# Autodesk Inventor assembly: platform
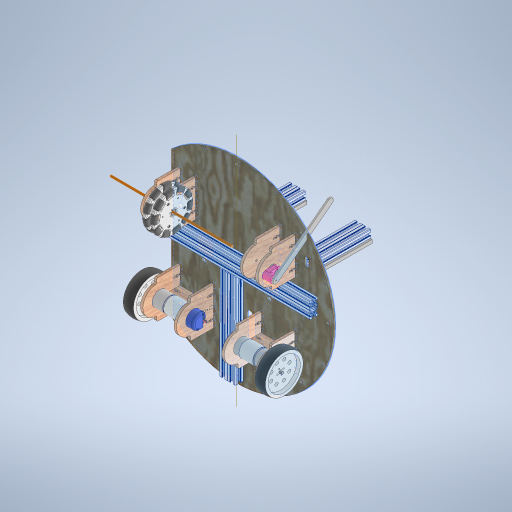
[picture p0: Inventor's stored thumbnail of the model, 512x512]
Saved by Autodesk Inventor 2023.1 (Build 271208000, 208)
## iProperties
Created: 2023-03-13
Part Number: platform
Document SubType Name: Assembly
Designer: User
Author: User
## Documents named in this file (24)
- C:\Users\DELL\reposGitHub\Cheburashka\Cheburashka_construction\platform\platform.iam
- C:\Users\DELL\reposGitHub\Cheburashka\Cheburashka_construction\platform\Osn. platform.ipt
- C:\Users\DELL\reposGitHub\Cheburashka\Cheburashka_construction\platform\motor1.ipt
- C:\Users\DELL\reposGitHub\Cheburashka\Cheburashka_construction\platform\motor2.ipt
- C:\Users\DELL\reposGitHub\Cheburashka\Cheburashka_construction\platform\motor3.ipt
- C:\Users\DELL\reposGitHub\Cheburashka\Cheburashka_construction\platform\wheel1.ipt
- C:\Users\DELL\reposGitHub\Cheburashka\Cheburashka_construction\platform\44260_txm torquenado dc motor_MIR2.ipt
- C:\Users\DELL\reposGitHub\Cheburashka\Cheburashka_construction\platform\36466_txm-4 inch omni wheel.ipt
- C:\Users\DELL\reposGitHub\Cheburashka\Cheburashka_construction\platform\39055_txm-4 inch wheel_MIR1.ipt
- C:\Users\DELL\reposGitHub\Cheburashka\Cheburashka_construction\platform\motor1_MIR3.ipt
- C:\Users\DELL\reposGitHub\Cheburashka\Cheburashka_construction\platform\motor2_MIR3.ipt
- C:\Users\DELL\reposGitHub\Cheburashka\Cheburashka_construction\platform\motor3_MIR3.ipt
- C:\Users\DELL\reposGitHub\Cheburashka\Cheburashka_construction\platform\44260_txm torquenado dc motor_MIR2_MIR.ipt
- C:\Users\DELL\reposGitHub\Cheburashka\Cheburashka_construction\platform\wheel1_MIR.ipt
- C:\Users\DELL\reposGitHub\Cheburashka\Cheburashka_construction\platform\36466_txm-4 inch omni wheel_MIR2.ipt
- C:\Users\DELL\reposGitHub\Cheburashka\Cheburashka_construction\platform\39055_txm-4 inch wheel_MIR1_MIR.ipt
- C:\Users\DELL\reposGitHub\Cheburashka\Cheburashka_construction\platform\кривошип.ipt
- C:\Users\DELL\reposGitHub\Cheburashka\Cheburashka_construction\platform\ось колес2.ipt
- C:\Users\DELL\reposGitHub\Cheburashka\Cheburashka_construction\platform\akfytw2.ipt
- C:\Users\DELL\reposGitHub\Cheburashka\Cheburashka_construction\platform\подшипник2.ipt
- C:\Users\DELL\reposGitHub\Cheburashka\Cheburashka_construction\platform\шатун22.ipt
- C:\Users\DELL\reposGitHub\Cheburashka\Cheburashka_construction\platform\канал_проводов.ipt
- C:\Users\DELL\reposGitHub\Cheburashka\Cheburashka_construction\platform\обр_профиль.ipt
- C:\Users\DELL\reposGitHub\Cheburashka\Cheburashka_construction\platform\обр_профиль2.ipt
## Components (29 placed, 23 different names)
1. Osn. platform:1 — Совмещение:1, Совмещение:2, Совмещение:5, Совмещение:8, Совмещение:29, Совмещение:30, Совмещение:31, Совмещение:32, Совмещение:33, Совмещение:34, Совмещение:97, Совмещение:98, Совмещение:114, Совмещение:115, Совмещение:117, Совмещение:118, Совмещение:125, Совмещение:126, Совмещение:127, Совмещение:128, Совмещение:129, Совмещение:130, Совмещение:131, Совмещение:132, Совмещение:133, Совмещение:137, Совмещение:138, Совмещение:140, Совмещение:141, Совмещение:142, Совмещение:143, Совмещение:144, Совмещение:145, Совмещение:146, Совмещение:147
2. motor1:1 — Совмещение:2, Совмещение:31, Совмещение:32
3. motor2:1 — Совмещение:5, Совмещение:29, Совмещение:30
4. motor3:1 — Совмещение:8, Совмещение:11, Совмещение:12, Совмещение:22, Совмещение:33, Совмещение:34
5. 44260_txm torquenado dc motor_MIR2:1 — Совмещение:11, Совмещение:12, Совмещение:21
6. wheel1:1 — Совмещение:101, Совмещение:140, Совмещение:141
7. wheel1:2 — Совмещение:97, Совмещение:98
8. 36466_txm-4 inch omni wheel:1 — Совмещение:102
9. 39055_txm-4 inch wheel_MIR1:1 — Совмещение:21, Совмещение:22
10. motor1_MIR3:1 — Совмещение:146, Совмещение:147
11. motor2_MIR3:1 — Совмещение:144, Совмещение:145
12. motor3_MIR3:1 — Совмещение:109, Совмещение:110, Совмещение:111, Совмещение:142, Совмещение:143
13. 44260_txm torquenado dc motor_MIR2_MIR:1 — Совмещение:28, Совмещение:109, Совмещение:110
14. wheel1_MIR:1 — Совмещение:117, Совмещение:118
15. wheel1_MIR:2 — Совмещение:87, Совмещение:113, Совмещение:114, Совмещение:115
16. 36466_txm-4 inch omni wheel_MIR2:1 — Совмещение:112, Совмещение:113
17. 39055_txm-4 inch wheel_MIR1_MIR:1 — Совмещение:28, Совмещение:111
18. кривошип:1 — Совмещение:90, Совмещение:91, Совмещение:92, Совмещение:93, Совмещение:96
19. ось колес2:1 — Совмещение:87, Совмещение:89, Совмещение:102, Совмещение:112
20. akfytw2:1 — Совмещение:89, Совмещение:90, Совмещение:91, Совмещение:101
21. подшипник2:1 — Совмещение:92, Совмещение:93, Совмещение:94
22. подшипник2:2 — Совмещение:94, Совмещение:95
23. шатун22:1 — Совмещение:95, Совмещение:96
24. канал_проводов:1 — Совмещение:125, Совмещение:126
25. канал_проводов:2 — Совмещение:127, Совмещение:128
26. обр_профиль:1 — Совмещение:129, Совмещение:130, Совмещение:131
27. обр_профиль:2 — Совмещение:132, Совмещение:133, Совмещение:135, Совмещение:136
28. обр_профиль2:1 — Совмещение:135, Совмещение:136, Совмещение:139
29. обр_профиль:3 — Совмещение:137, Совмещение:138, Совмещение:139
## Relationships (59: Mate 59)
- Совмещение:1 [Mate]: Osn. platform:1
- Совмещение:2 [Mate]: Osn. platform:1 ↔ motor1:1
- Совмещение:5 [Mate]: Osn. platform:1 ↔ motor2:1
- Совмещение:8 [Mate]: Osn. platform:1 ↔ motor3:1
- Совмещение:11 [Mate]: motor3:1 ↔ 44260_txm torquenado dc motor_MIR2:1
- Совмещение:12 [Mate]: motor3:1 ↔ 44260_txm torquenado dc motor_MIR2:1
- Совмещение:21 [Mate]: 44260_txm torquenado dc motor_MIR2:1 ↔ 39055_txm-4 inch wheel_MIR1:1
- Совмещение:22 [Mate] (15 mm): motor3:1 ↔ 39055_txm-4 inch wheel_MIR1:1
- Совмещение:28 [Mate]: 44260_txm torquenado dc motor_MIR2_MIR:1 ↔ 39055_txm-4 inch wheel_MIR1_MIR:1
- Совмещение:29 [Mate]: Osn. platform:1 ↔ motor2:1
- Совмещение:30 [Mate]: Osn. platform:1 ↔ motor2:1
- Совмещение:31 [Mate]: Osn. platform:1 ↔ motor1:1
- Совмещение:32 [Mate]: Osn. platform:1 ↔ motor1:1
- Совмещение:33 [Mate]: Osn. platform:1 ↔ motor3:1
- Совмещение:34 [Mate]: Osn. platform:1 ↔ motor3:1
- Совмещение:87 [Mate]: wheel1_MIR:2 ↔ ось колес2:1
- Совмещение:89 [Mate]: ось колес2:1 ↔ akfytw2:1
- Совмещение:90 [Mate]: кривошип:1 ↔ akfytw2:1
- Совмещение:91 [Mate]: кривошип:1 ↔ akfytw2:1
- Совмещение:92 [Mate]: кривошип:1 ↔ подшипник2:1
- Совмещение:93 [Mate]: кривошип:1 ↔ подшипник2:1
- Совмещение:94 [Mate]: подшипник2:1 ↔ подшипник2:2
- Совмещение:95 [Mate]: подшипник2:2 ↔ шатун22:1
- Совмещение:96 [Mate] (2 mm): кривошип:1 ↔ шатун22:1
- Совмещение:97 [Mate]: Osn. platform:1 ↔ wheel1:2
- Совмещение:98 [Mate]: Osn. platform:1 ↔ wheel1:2
- Совмещение:101 [Mate]: wheel1:1 ↔ akfytw2:1
- Совмещение:102 [Mate]: 36466_txm-4 inch omni wheel:1 ↔ ось колес2:1
- Совмещение:109 [Mate]: motor3_MIR3:1 ↔ 44260_txm torquenado dc motor_MIR2_MIR:1
- Совмещение:110 [Mate]: motor3_MIR3:1 ↔ 44260_txm torquenado dc motor_MIR2_MIR:1
- Совмещение:111 [Mate] (5 mm): motor3_MIR3:1 ↔ 39055_txm-4 inch wheel_MIR1_MIR:1
- Совмещение:112 [Mate]: 36466_txm-4 inch omni wheel_MIR2:1 ↔ ось колес2:1
- Совмещение:113 [Mate] (10 mm): wheel1_MIR:2 ↔ 36466_txm-4 inch omni wheel_MIR2:1
- Совмещение:114 [Mate]: Osn. platform:1 ↔ wheel1_MIR:2
- Совмещение:115 [Mate]: Osn. platform:1 ↔ wheel1_MIR:2
- Совмещение:117 [Mate]: Osn. platform:1 ↔ wheel1_MIR:1
- Совмещение:118 [Mate]: Osn. platform:1 ↔ wheel1_MIR:1
- Совмещение:125 [Mate]: Osn. platform:1 ↔ канал_проводов:1
- Совмещение:126 [Mate]: Osn. platform:1 ↔ канал_проводов:1
- Совмещение:127 [Mate]: Osn. platform:1 ↔ канал_проводов:2
- Совмещение:128 [Mate]: Osn. platform:1 ↔ канал_проводов:2
- Совмещение:129 [Mate]: Osn. platform:1 ↔ обр_профиль:1
- Совмещение:130 [Mate]: Osn. platform:1 ↔ обр_профиль:1
- Совмещение:131 [Mate]: Osn. platform:1 ↔ обр_профиль:1
- Совмещение:132 [Mate]: Osn. platform:1 ↔ обр_профиль:2
- Совмещение:133 [Mate]: Osn. platform:1 ↔ обр_профиль:2
- Совмещение:135 [Mate] (99.253 mm): обр_профиль:2 ↔ обр_профиль2:1
- Совмещение:136 [Mate]: обр_профиль:2 ↔ обр_профиль2:1
- Совмещение:137 [Mate]: Osn. platform:1 ↔ обр_профиль:3
- Совмещение:138 [Mate] (4.43 mm): Osn. platform:1 ↔ обр_профиль:3
- Совмещение:139 [Mate]: обр_профиль2:1 ↔ обр_профиль:3
- Совмещение:140 [Mate]: Osn. platform:1 ↔ wheel1:1
- Совмещение:141 [Mate]: Osn. platform:1 ↔ wheel1:1
- Совмещение:142 [Mate]: Osn. platform:1 ↔ motor3_MIR3:1
- Совмещение:143 [Mate]: Osn. platform:1 ↔ motor3_MIR3:1
- Совмещение:144 [Mate]: Osn. platform:1 ↔ motor2_MIR3:1
- Совмещение:145 [Mate]: Osn. platform:1 ↔ motor2_MIR3:1
- Совмещение:146 [Mate]: Osn. platform:1 ↔ motor1_MIR3:1
- Совмещение:147 [Mate]: Osn. platform:1 ↔ motor1_MIR3:1
